# Autodesk Inventor assembly: assembled
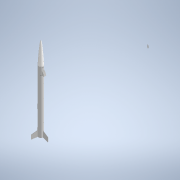
[picture p0: Inventor's stored thumbnail of the model, 180x180]
Saved by Autodesk Inventor 2020.3 (Build 243373000, 373)
## iProperties
Created: 2021-03-15
Part Number: assembled
Document SubType Name: Assembly
Designer: 0x6f736f646f
Author: 0x6f736f646f
## Documents named in this file (10)
- C:\Users\0x6f736f646f\OneDrive\Documents\Nakuja\airframev1\Design\assembled.iam
- C:\Users\0x6f736f646f\OneDrive\Documents\Nakuja\airframev1\Design\noseAssembly.iam
- C:\Users\0x6f736f646f\OneDrive\Documents\Nakuja\airframev1\Design\electronicsbay.ipt
- C:\Users\0x6f736f646f\OneDrive\Documents\Nakuja\airframev1\Design\extraTube.ipt
- C:\Users\0x6f736f646f\OneDrive\Documents\Nakuja\airframev1\Design\launchlug.ipt
- C:\Users\0x6f736f646f\OneDrive\Documents\Nakuja\airframev1\Design\payloadchamber.ipt
- C:\Users\0x6f736f646f\OneDrive\Documents\Nakuja\airframev1\Design\tail.ipt
- C:\Users\0x6f736f646f\OneDrive\Documents\Nakuja\airframev1\Design\motor-mount-bottom.ipt
- C:\Users\0x6f736f646f\OneDrive\Documents\Nakuja\airframev1\Design\picameraholder.ipt
- C:\Users\0x6f736f646f\OneDrive\Documents\Nakuja\airframev1\Design\servoarm.ipt
## Components (11 placed, 9 different names)
1. noseAssembly:1 [sub-assembly] — Insert:1
2. electronicsbay:1 — Mate:1, Mate:2
3. extraTube:1 — Insert:3, Insert:4
4. launchlug:1 — Mate:7
5. motor-mount-bottom:1 — Mate:3, Mate:4
6. payloadchamber:1 — Insert:1, Insert:2, Mate:1, Mate:2, Mate:5, Mate:6, Tangent:1
7. picameraholder:1 — Mate:5, Mate:6
8. servoarm:1 — Tangent:1
9. launchlug:2 — Mate:7, Mate:8, Mate:9
10. extraTube:2 — Insert:2, Insert:3
11. tail:1 — Insert:4, Mate:3, Mate:4, Mate:8, Mate:9
## Relationships (14: Mate 9, Insert 4, Tangent 1)
- Insert:1: noseAssembly:1 ↔ payloadchamber:1
- Insert:2: payloadchamber:1 ↔ extraTube:2
- Insert:3: extraTube:1 ↔ extraTube:2
- Mate:1: electronicsbay:1 ↔ payloadchamber:1
- Mate:2: electronicsbay:1 ↔ payloadchamber:1
- Insert:4: extraTube:1 ↔ tail:1
- Mate:3: motor-mount-bottom:1 ↔ tail:1
- Mate:4: motor-mount-bottom:1 ↔ tail:1
- Mate:5: payloadchamber:1 ↔ picameraholder:1
- Mate:6: payloadchamber:1 ↔ picameraholder:1
- Mate:7: launchlug:1 ↔ launchlug:2
- Mate:8 (33.6 mm): launchlug:2 ↔ tail:1
- Mate:9: launchlug:2 ↔ tail:1
- Tangent:1: payloadchamber:1 ↔ servoarm:1
